# Autodesk Inventor assembly: Ensamble_sensor
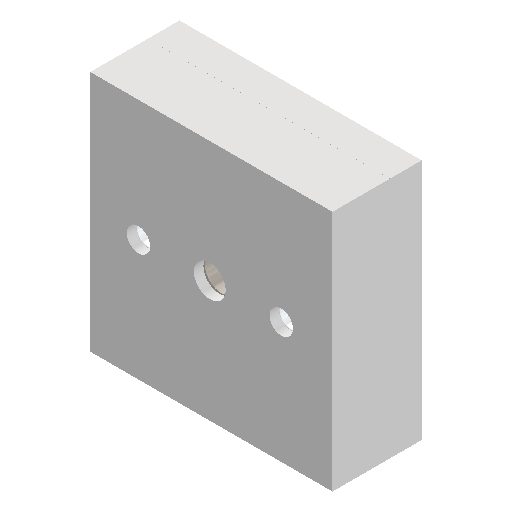
[picture p0: Inventor's stored thumbnail of the model, 512x512]
Saved by Autodesk Inventor 2025 (Build 290162000, 162)
## iProperties
Created: 2026-02-02
Part Number: Ensamble_sensor
Document SubType Name: Assembly
Designer: HP
Author: HP
## Documents named in this file (4)
- C:\Users\HP\Desktop\CAD\Ensamble_sensor.iam
- C:\Users\HP\Desktop\CAD\3D_PCB3_2026-01-02\3D_PCB3_2026-01-02.iam
- C:\Users\HP\Desktop\CAD\TORNILLO ALLEN CABEZA PLANA M3x0.5x6\sensor_estructura.ipt
- C:\Users\HP\Desktop\CAD\sensor_chumacera.iam
## Components (3 placed, 3 different names)
1. 3D_PCB3_2026-01-02:1 [sub-assembly] — Nivelación:1
2. sensor_estructura:1 — Nivelación:1
3. sensor_chumacera:1 [sub-assembly]
## Relationships (1: Flush 1)
- Nivelación:1 [Flush]: 3D_PCB3_2026-01-02:1 ↔ sensor_estructura:1
